# Autodesk Inventor assembly: warehouse_version_2
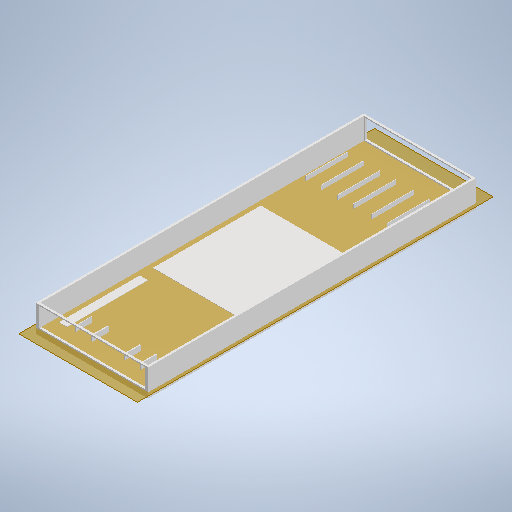
[picture p0: Inventor's stored thumbnail of the model, 512x512]
Saved by Autodesk Inventor 2025 (Build 290162000, 162)
## iProperties
Created: 2025-05-08
Part Number: warehouse_version_2
Document SubType Name: Assembly
Designer: Ennis
Author: Ennis
## Documents named in this file (3)
- C:\Users\ennis\Documents\Financien_Werk_OV\my_works\Courses TM\2024-2025\Semester 2\Practise Entreprise\server\ros_ws\src\robot_gz_startup\meshes\warehouse\warehouse_version_2.iam
- C:\Users\ennis\Documents\base.ipt
- C:\Users\ennis\Documents\inside.ipt
## Components (2 placed, 2 different names)
1. base:1 — Flush:1, Flush:2, Flush:3, Flush:4, Flush:5
2. inside:1 — Flush:1, Flush:2, Flush:3, Flush:4, Flush:5
## Relationships (5: Flush 5)
- Flush:1: base:1 ↔ inside:1
- Flush:2: base:1 ↔ inside:1
- Flush:3: base:1 ↔ inside:1
- Flush:4: base:1 ↔ inside:1
- Flush:5: base:1 ↔ inside:1
